# Autodesk Inventor assembly: assembled-antenna
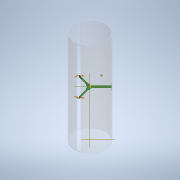
[picture p0: Inventor's stored thumbnail of the model, 180x180]
Saved by Autodesk Inventor 2021 (Build 250183000, 183)
## iProperties
Created: 2020-09-03
Part Number: assembled-antenna
Document SubType Name: Assembly
Designer: dsouthall
Author: dsouthall
## Documents named in this file (7)
- C:\Users\dsouthall\OneDrive - The University of Chicago\Hpol\Model 8 in\assembled-antenna.iam
- C:\Users\dsouthall\OneDrive - The University of Chicago\Hpol\Model 8 in\assembled-feed.iam
- C:\Users\dsouthall\OneDrive - The University of Chicago\Hpol\Model 8 in\source\my can\can.ipt
- C:\Users\dsouthall\OneDrive - The University of Chicago\Hpol\Model 8 in\source\92141A003_TYPE 18-8 STAINLESS STEEL FLAT WASHER\92141A003_TYPE 18-8 STAINLESS STEEL FLAT WASHER.ipt
- C:\Users\dsouthall\OneDrive - The University of Chicago\Hpol\Model 8 in\source\96877A118_18-8 SS 82 DEG FLAT HEAD PHIL MACHINE SCREW\96877A118_18-8 SS 82 DEG FLAT HEAD PHIL MACHINE SCREW.ipt
- C:\Users\dsouthall\OneDrive - The University of Chicago\Hpol\Model 8 in\source\91841A003_TYPE 18-8 STAINLESS STEEL HEX NUT\91841A003_TYPE 18-8 STAINLESS STEEL HEX NUT.ipt
- C:\Users\dsouthall\OneDrive - The University of Chicago\Hpol\Model 8 in\source\my_faceplate.ipt
## Components (22 placed, 6 different names)
1. can:1 — Insert:19, Insert:20, Insert:25, Insert:26, Insert:27, Insert:28, Insert:37, Insert:38, Mate:3, Mate:4, Mate:5
2. my_faceplate:1 — Insert:37, Angle:3
3. my_faceplate:2 — Insert:38, Angle:3
4. assembled-feed:1 [sub-assembly] — Mate:3, Mate:5
5. 96877A118_18-8 SS 82 DEG FLAT HEAD PHIL MACHINE SCREW:3 — Insert:26, Insert:35
6. 96877A118_18-8 SS 82 DEG FLAT HEAD PHIL MACHINE SCREW:4 — Insert:25, Insert:33
7. 96877A118_18-8 SS 82 DEG FLAT HEAD PHIL MACHINE SCREW:5 — Insert:28, Insert:29
8. 96877A118_18-8 SS 82 DEG FLAT HEAD PHIL MACHINE SCREW:6 — Insert:27, Insert:30
9. 92141A003_TYPE 18-8 STAINLESS STEEL FLAT WASHER:9 — Insert:30, Insert:32
10. 92141A003_TYPE 18-8 STAINLESS STEEL FLAT WASHER:10 — Insert:29, Insert:31
11. 92141A003_TYPE 18-8 STAINLESS STEEL FLAT WASHER:11 — Insert:33, Insert:34
12. 92141A003_TYPE 18-8 STAINLESS STEEL FLAT WASHER:12 — Insert:35, Insert:36
13. 91841A003_TYPE 18-8 STAINLESS STEEL HEX NUT:3 — Insert:36
14. 91841A003_TYPE 18-8 STAINLESS STEEL HEX NUT:4 — Insert:34
15. 91841A003_TYPE 18-8 STAINLESS STEEL HEX NUT:5 — Insert:31
16. 91841A003_TYPE 18-8 STAINLESS STEEL HEX NUT:6 — Insert:32
17. 96877A118_18-8 SS 82 DEG FLAT HEAD PHIL MACHINE SCREW:1 — Insert:19, Insert:21
18. 96877A118_18-8 SS 82 DEG FLAT HEAD PHIL MACHINE SCREW:2 — Insert:20, Insert:23
19. 92141A003_TYPE 18-8 STAINLESS STEEL FLAT WASHER:7 — Insert:23, Insert:24
20. 92141A003_TYPE 18-8 STAINLESS STEEL FLAT WASHER:8 — Insert:21, Insert:22
21. 91841A003_TYPE 18-8 STAINLESS STEEL HEX NUT:1 — Insert:24
22. 91841A003_TYPE 18-8 STAINLESS STEEL HEX NUT:2 — Insert:22
## Relationships (24: Insert 20, Mate 3, Angle 1)
- Insert:19: can:1 ↔ 96877A118_18-8 SS 82 DEG FLAT HEAD PHIL MACHINE SCREW:1
- Insert:20: can:1 ↔ 96877A118_18-8 SS 82 DEG FLAT HEAD PHIL MACHINE SCREW:2
- Insert:21 (-2.54 mm): 96877A118_18-8 SS 82 DEG FLAT HEAD PHIL MACHINE SCREW:1 ↔ 92141A003_TYPE 18-8 STAINLESS STEEL FLAT WASHER:8
- Insert:22: 92141A003_TYPE 18-8 STAINLESS STEEL FLAT WASHER:8 ↔ 91841A003_TYPE 18-8 STAINLESS STEEL HEX NUT:2
- Insert:23 (-2.54 mm): 96877A118_18-8 SS 82 DEG FLAT HEAD PHIL MACHINE SCREW:2 ↔ 92141A003_TYPE 18-8 STAINLESS STEEL FLAT WASHER:7
- Insert:24: 92141A003_TYPE 18-8 STAINLESS STEEL FLAT WASHER:7 ↔ 91841A003_TYPE 18-8 STAINLESS STEEL HEX NUT:1
- Insert:25: can:1 ↔ 96877A118_18-8 SS 82 DEG FLAT HEAD PHIL MACHINE SCREW:4
- Insert:26: can:1 ↔ 96877A118_18-8 SS 82 DEG FLAT HEAD PHIL MACHINE SCREW:3
- Insert:27: can:1 ↔ 96877A118_18-8 SS 82 DEG FLAT HEAD PHIL MACHINE SCREW:6
- Insert:28: can:1 ↔ 96877A118_18-8 SS 82 DEG FLAT HEAD PHIL MACHINE SCREW:5
- Insert:29 (-2.54 mm): 96877A118_18-8 SS 82 DEG FLAT HEAD PHIL MACHINE SCREW:5 ↔ 92141A003_TYPE 18-8 STAINLESS STEEL FLAT WASHER:10
- Insert:30 (-2.54 mm): 96877A118_18-8 SS 82 DEG FLAT HEAD PHIL MACHINE SCREW:6 ↔ 92141A003_TYPE 18-8 STAINLESS STEEL FLAT WASHER:9
- Insert:31: 92141A003_TYPE 18-8 STAINLESS STEEL FLAT WASHER:10 ↔ 91841A003_TYPE 18-8 STAINLESS STEEL HEX NUT:5
- Insert:32: 92141A003_TYPE 18-8 STAINLESS STEEL FLAT WASHER:9 ↔ 91841A003_TYPE 18-8 STAINLESS STEEL HEX NUT:6
- Insert:33 (-2.54 mm): 96877A118_18-8 SS 82 DEG FLAT HEAD PHIL MACHINE SCREW:4 ↔ 92141A003_TYPE 18-8 STAINLESS STEEL FLAT WASHER:11
- Insert:34: 92141A003_TYPE 18-8 STAINLESS STEEL FLAT WASHER:11 ↔ 91841A003_TYPE 18-8 STAINLESS STEEL HEX NUT:4
- Insert:35 (-2.54 mm): 96877A118_18-8 SS 82 DEG FLAT HEAD PHIL MACHINE SCREW:3 ↔ 92141A003_TYPE 18-8 STAINLESS STEEL FLAT WASHER:12
- Insert:36: 92141A003_TYPE 18-8 STAINLESS STEEL FLAT WASHER:12 ↔ 91841A003_TYPE 18-8 STAINLESS STEEL HEX NUT:3
- Insert:37: can:1 ↔ my_faceplate:1
- Insert:38 (-9.652 mm): can:1 ↔ my_faceplate:2
- Angle:3 (0 deg): my_faceplate:1 ↔ my_faceplate:2
- Mate:3: can:1 ↔ assembled-feed:1
- Mate:4 (600 mm): can:1
- Mate:5 (300 mm): can:1 ↔ assembled-feed:1
